# Autodesk Inventor assembly: Робот_ЕТЗ
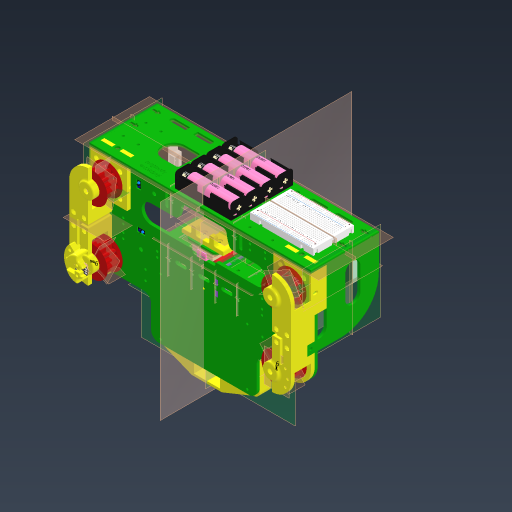
[picture p0: Inventor's stored thumbnail of the model, 512x512]
Saved by Autodesk Inventor 2023.2 (Build 272271030, 271C)
## iProperties
Created: 2025-12-08
Part Number: Робот_ЕТЗ
Document SubType Name: Assembly
Designer: Олег Коноваленко
Author: Олег Коноваленко
## Documents named in this file (25)
- D:\VSOSH_IT_Robotics_ETZ\ETZ\Сonstruction\Робот_ЕТЗ.iam
- D:\VSOSH_IT_Robotics_ETZ\ETZ\Сonstruction\Nema 17.ipt
- D:\VSOSH_IT_Robotics_ETZ\ETZ\Сonstruction\Передняя_крышка.ipt
- D:\VSOSH_IT_Robotics_ETZ\ETZ\Сonstruction\Print\Вал_ведомых_шестерн.ipt
- D:\VSOSH_IT_Robotics_ETZ\ETZ\Сonstruction\Крепление_ведомых_шестерн.ipt
- D:\VSOSH_IT_Robotics_ETZ\ETZ\Сonstruction\Фланцевая_муфта.ipt
- D:\VSOSH_IT_Robotics_ETZ\ETZ\Сonstruction\Вал_ведущих_шестерн.ipt
- D:\VSOSH_IT_Robotics_ETZ\ETZ\Сonstruction\Ведомая_шестерня.ipt
- D:\VSOSH_IT_Robotics_ETZ\ETZ\Сonstruction\Ведущая_шеестерня.ipt
- D:\VSOSH_IT_Robotics_ETZ\ETZ\Сonstruction\Крепление_ведомых_шестерн_MIR1.ipt
- D:\VSOSH_IT_Robotics_ETZ\ETZ\Сonstruction\TCRT5000.ipt
- D:\VSOSH_IT_Robotics_ETZ\ETZ\Сonstruction\Крепление_TCRT.ipt
- D:\VSOSH_IT_Robotics_ETZ\ETZ\Сonstruction\AS5048A Magnetic Encoder - B.ipt
- D:\VSOSH_IT_Robotics_ETZ\ETZ\Сonstruction\Выступ_под_крепление_маркера.ipt
- D:\VSOSH_IT_Robotics_ETZ\ETZ\Сonstruction\Рёбра_жёсткости.ipt
- D:\VSOSH_IT_Robotics_ETZ\ETZ\Сonstruction\Плата.ipt
- D:\VSOSH_IT_Robotics_ETZ\ETZ\Сonstruction\Стойка.ipt
- D:\VSOSH_IT_Robotics_ETZ\ETZ\Сonstruction\Фанерка_аккумуляторов.ipt
- D:\VSOSH_IT_Robotics_ETZ\ETZ\Сonstruction\Holder 18650 (4 cell)_series_pink.ipt
- D:\VSOSH_IT_Robotics_ETZ\ETZ\Сonstruction\Крышка_электроники.ipt
- D:\VSOSH_IT_Robotics_ETZ\ETZ\Сonstruction\Breadboard 400.ipt
- D:\VSOSH_IT_Robotics_ETZ\ETZ\Сonstruction\Крепление_энкодера.ipt
- D:\VSOSH_IT_Robotics_ETZ\ETZ\Сonstruction\Модуль_маркера.iam
- D:\VSOSH_IT_Robotics_ETZ\ETZ\Сonstruction\Рёбра_жёсткости_индивиды.ipt
- D:\VSOSH_IT_Robotics_ETZ\ETZ\Сonstruction\дополнительное_ребро_жёсткости.ipt
## Components (41 placed, 24 different names)
1. Nema 17:1 — Совмещение:78, Заподлицо:26, Угол:1
2. Передняя_крышка:1 — Совмещение:79, Совмещение:80, Совмещение:81, Заподлицо:28, Совмещение:82, Совмещение:95, Совмещение:96, Совмещение:98, Совмещение:99, Заподлицо:38, Совмещение:104, Совмещение:105, Заподлицо:42, Совмещение:109, Заподлицо:44, Заподлицо:45, Совмещение:110, Совмещение:111, Совмещение:112, Совмещение:113, Совмещение:120, Заподлицо:49, Совмещение:123, Совмещение:124, Совмещение:130, Заподлицо:57, Совмещение:143, Совмещение:144, Совмещение:145, Совмещение:146, Совмещение:147, Совмещение:148
3. Вал_ведомых_шестерн:1 — Совмещение:85
4. Крепление_ведомых_шестерн:1 — Совмещение:64, Совмещение:68, Совмещение:70, Заподлицо:23, Совмещение:73, Совмещение:79, Совмещение:80, Угол:1, Совмещение:139, Заподлицо:65, Совмещение:140, Совмещение:157, Совмещение:158
5. Фланцевая_муфта:1 — Совмещение:64, Совмещение:65, Совмещение:68, Совмещение:74, Совмещение:78, Заподлицо:26
6. Вал_ведущих_шестерн:1 — Совмещение:70, Заподлицо:23
7. Ведомая_шестерня:1 — Совмещение:85, Совмещение:157, Совмещение:158
8. Ведущая_шестерня:2 — Совмещение:65, Совмещение:73, Совмещение:74
9. Крепление_ведомых_шестерн_MIR1:1 — Совмещение:81, Заподлицо:28, Совмещение:82, Совмещение:84, Совмещение:86, Совмещение:87, Угол:2, Совмещение:119, Заподлицо:47, Заподлицо:48, Совмещение:155, Совмещение:156
10. Ведущая_шестерня:3 — Совмещение:86, Совмещение:87, Совмещение:88, Совмещение:91
11. Ведомая_шестерня:2 — Совмещение:84, Совмещение:156
12. Nema 17:2 — Совмещение:90, Заподлицо:29, Угол:2
13. Фланцевая_муфта:2 — Совмещение:88, Совмещение:90, Заподлицо:29, Совмещение:91
14. TCRT5000:1 — Совмещение:92, Заподлицо:30, Заподлицо:31
15. Крепление_TCRT:1 — Совмещение:92, Заподлицо:30, Заподлицо:31, Совмещение:95, Заподлицо:43, Заподлицо:46
16. TCRT5000:2
17. Крепление_TCRT:2 — Совмещение:96, Заподлицо:42, Заподлицо:43
18. AS5048A Magnetic Encoder - B:1 — Совмещение:136, Совмещение:137, Совмещение:138
19. Выступ_под_крепление_маркера:1 — Совмещение:98, Совмещение:99, Заподлицо:38, Совмещение:106, Совмещение:107, Совмещение:108, Заподлицо:41, Заподлицо:46, Совмещение:141, Заподлицо:66, Совмещение:142
20. Рёбра_жёсткости:3 — Совмещение:104, Совмещение:107, Совмещение:108
21. Рёбра_жёсткости:4 — Совмещение:105, Совмещение:106, Заподлицо:41
22. Плата:1 — Совмещение:109, Заподлицо:44, Заподлицо:45, Совмещение:114, Совмещение:115, Совмещение:116, Совмещение:117, Заподлицо:59, Заподлицо:60, Заподлицо:61, Заподлицо:62
23. Стойка:1 — Совмещение:110, Совмещение:115, Заподлицо:61
24. Стойка:2 — Совмещение:111, Совмещение:116, Заподлицо:62
25. Стойка:3 — Совмещение:112, Совмещение:117, Заподлицо:59
26. Стойка:4 — Совмещение:113, Совмещение:114, Заподлицо:60
27. Фанерка_аккумуляторов:1 — Совмещение:119, Заподлицо:47, Заподлицо:48, Совмещение:121, Совмещение:122, Совмещение:131, Заподлицо:63, Заподлицо:64, Совмещение:152, Заподлицо:73, Заподлицо:74, Заподлицо:75, Совмещение:154, Заподлицо:76, Заподлицо:77
28. Рёбра_жёсткости:5 — Совмещение:120, Совмещение:121, Заподлицо:49
29. Рёбра_жёсткости:6 — Совмещение:122, Совмещение:123, Совмещение:124
30. Holder 18650 (4 cell)_series_pink:1 — Заподлицо:69, Совмещение:149, Заподлицо:72
31. Holder 18650 (4 cell)_series_pink:3 — Заподлицо:68, Заподлицо:69, Совмещение:150, Совмещение:151, Заподлицо:70, Заподлицо:71, Совмещение:153
32. Holder 18650 (4 cell)_series_pink:4 — Заподлицо:67, Заподлицо:68, Совмещение:149, Совмещение:150, Заподлицо:71, Заподлицо:72
33. Крышка_электроники:1 — Совмещение:130, Заподлицо:57
34. Breadboard 400:1 — Совмещение:131, Заподлицо:63, Заподлицо:64
35. Крепление_энкодера:1 — Совмещение:136, Совмещение:137, Совмещение:138, Совмещение:139, Заподлицо:65, Совмещение:140
36. Модуль_маркера:1 [sub-assembly] — Совмещение:141, Заподлицо:66, Совмещение:142
37. Рёбра_жёсткости_индивиды:1 — Совмещение:143, Совмещение:147, Совмещение:148
38. Рёбра_жёсткости_индивиды:2 — Совмещение:144, Совмещение:145, Совмещение:146
39. Holder 18650 (4 cell)_series_pink:5 — Заподлицо:67, Совмещение:151, Заподлицо:70, Совмещение:152, Заподлицо:73
40. дополнительное_ребро_жёсткости:1 — Заподлицо:74, Заподлицо:75, Совмещение:154
41. дополнительное_ребро_жёсткости:2 — Совмещение:155, Заподлицо:76, Заподлицо:77
## Relationships (109: Mate 69, Flush 38, Angle 2)
- Совмещение:64 [Mate]: Крепление_ведомых_шестерн:1 ↔ Фланцевая_муфта:1
- Совмещение:65 [Mate]: Фланцевая_муфта:1 ↔ Ведущая_шестерня:2
- Совмещение:68 [Mate]: Крепление_ведомых_шестерн:1 ↔ Фланцевая_муфта:1
- Совмещение:70 [Mate]: Крепление_ведомых_шестерн:1 ↔ Вал_ведущих_шестерн:1
- Заподлицо:23 [Flush]: Крепление_ведомых_шестерн:1 ↔ Вал_ведущих_шестерн:1
- Совмещение:73 [Mate] (0.5 mm): Крепление_ведомых_шестерн:1 ↔ Ведущая_шестерня:2
- Совмещение:74 [Mate]: Фланцевая_муфта:1 ↔ Ведущая_шестерня:2
- Совмещение:78 [Mate]: Nema 17:1 ↔ Фланцевая_муфта:1
- Заподлицо:26 [Flush]: Nema 17:1 ↔ Фланцевая_муфта:1
- Совмещение:79 [Mate]: Передняя_крышка:1 ↔ Крепление_ведомых_шестерн:1
- Совмещение:80 [Mate]: Передняя_крышка:1 ↔ Крепление_ведомых_шестерн:1
- Совмещение:81 [Mate]: Передняя_крышка:1 ↔ Крепление_ведомых_шестерн_MIR1:1
- Заподлицо:28 [Flush]: Передняя_крышка:1 ↔ Крепление_ведомых_шестерн_MIR1:1
- Совмещение:82 [Mate]: Передняя_крышка:1 ↔ Крепление_ведомых_шестерн_MIR1:1
- Совмещение:84 [Mate]: Крепление_ведомых_шестерн_MIR1:1 ↔ Ведомая_шестерня:2
- Совмещение:85 [Mate]: Вал_ведомых_шестерн:1 ↔ Ведомая_шестерня:1
- Совмещение:86 [Mate] (0.5 mm): Крепление_ведомых_шестерн_MIR1:1 ↔ Ведущая_шестерня:3
- Совмещение:87 [Mate]: Крепление_ведомых_шестерн_MIR1:1 ↔ Ведущая_шестерня:3
- Угол:1 [Angle] (0 deg): Nema 17:1 ↔ Крепление_ведомых_шестерн:1
- Совмещение:88 [Mate]: Ведущая_шестерня:3 ↔ Фланцевая_муфта:2
- Совмещение:90 [Mate]: Nema 17:2 ↔ Фланцевая_муфта:2
- Заподлицо:29 [Flush]: Nema 17:2 ↔ Фланцевая_муфта:2
- Совмещение:91 [Mate]: Ведущая_шестерня:3 ↔ Фланцевая_муфта:2
- Угол:2 [Angle] (0 deg): Крепление_ведомых_шестерн_MIR1:1 ↔ Nema 17:2
- Совмещение:92 [Mate]: TCRT5000:1 ↔ Крепление_TCRT:1
- Заподлицо:30 [Flush]: TCRT5000:1 ↔ Крепление_TCRT:1
- Заподлицо:31 [Flush]: TCRT5000:1 ↔ Крепление_TCRT:1
- [Mate]: TCRT5000:2 ↔ Крепление_TCRT:2
- [Flush]: TCRT5000:2 ↔ Крепление_TCRT:2
- [Flush]: TCRT5000:2 ↔ Крепление_TCRT:2
- Совмещение:95 [Mate]: Передняя_крышка:1 ↔ Крепление_TCRT:1
- Совмещение:96 [Mate]: Передняя_крышка:1 ↔ Крепление_TCRT:2
- Совмещение:98 [Mate]: Передняя_крышка:1 ↔ Выступ_под_крепление_маркера:1
- Совмещение:99 [Mate]: Передняя_крышка:1 ↔ Выступ_под_крепление_маркера:1
- Заподлицо:38 [Flush] (10 mm): Передняя_крышка:1 ↔ Выступ_под_крепление_маркера:1
- Совмещение:104 [Mate]: Передняя_крышка:1 ↔ Рёбра_жёсткости:3
- Совмещение:105 [Mate]: Передняя_крышка:1 ↔ Рёбра_жёсткости:4
- Совмещение:106 [Mate]: Выступ_под_крепление_маркера:1 ↔ Рёбра_жёсткости:4
- Совмещение:107 [Mate]: Выступ_под_крепление_маркера:1 ↔ Рёбра_жёсткости:3
- Совмещение:108 [Mate] (-14.25 mm): Выступ_под_крепление_маркера:1 ↔ Рёбра_жёсткости:3
- Заподлицо:41 [Flush] (14.25 mm): Выступ_под_крепление_маркера:1 ↔ Рёбра_жёсткости:4
- Заподлицо:42 [Flush] (10 mm): Передняя_крышка:1 ↔ Крепление_TCRT:2
- Заподлицо:43 [Flush]: Крепление_TCRT:1 ↔ Крепление_TCRT:2
- Совмещение:109 [Mate] (8 mm): Передняя_крышка:1 ↔ Плата:1
- Заподлицо:44 [Flush] (10 mm): Передняя_крышка:1 ↔ Плата:1
- Заподлицо:45 [Flush] (2.75 mm): Передняя_крышка:1 ↔ Плата:1
- Совмещение:110 [Mate]: Передняя_крышка:1 ↔ Стойка:1
- Совмещение:111 [Mate]: Передняя_крышка:1 ↔ Стойка:2
- Совмещение:112 [Mate]: Передняя_крышка:1 ↔ Стойка:3
- Совмещение:113 [Mate]: Передняя_крышка:1 ↔ Стойка:4
- Совмещение:114 [Mate]: Плата:1 ↔ Стойка:4
- Совмещение:115 [Mate]: Плата:1 ↔ Стойка:1
- Совмещение:116 [Mate]: Плата:1 ↔ Стойка:2
- Совмещение:117 [Mate]: Плата:1 ↔ Стойка:3
- Заподлицо:46 [Flush]: Крепление_TCRT:1 ↔ Выступ_под_крепление_маркера:1
- Совмещение:119 [Mate]: Крепление_ведомых_шестерн_MIR1:1 ↔ Фанерка_аккумуляторов:1
- Заподлицо:47 [Flush]: Крепление_ведомых_шестерн_MIR1:1 ↔ Фанерка_аккумуляторов:1
- Заподлицо:48 [Flush]: Крепление_ведомых_шестерн_MIR1:1 ↔ Фанерка_аккумуляторов:1
- Совмещение:120 [Mate]: Передняя_крышка:1 ↔ Рёбра_жёсткости:5
- Совмещение:121 [Mate]: Фанерка_аккумуляторов:1 ↔ Рёбра_жёсткости:5
- Заподлицо:49 [Flush] (40 mm): Передняя_крышка:1 ↔ Рёбра_жёсткости:5
- Совмещение:122 [Mate]: Фанерка_аккумуляторов:1 ↔ Рёбра_жёсткости:6
- Совмещение:123 [Mate]: Передняя_крышка:1 ↔ Рёбра_жёсткости:6
- Совмещение:124 [Mate] (40 mm): Передняя_крышка:1 ↔ Рёбра_жёсткости:6
- Совмещение:130 [Mate]: Передняя_крышка:1 ↔ Крышка_электроники:1
- Заподлицо:57 [Flush]: Передняя_крышка:1 ↔ Крышка_электроники:1
- Заподлицо:59 [Flush]: Плата:1 ↔ Стойка:3
- Заподлицо:60 [Flush]: Плата:1 ↔ Стойка:4
- Заподлицо:61 [Flush]: Плата:1 ↔ Стойка:1
- Заподлицо:62 [Flush]: Плата:1 ↔ Стойка:2
- Совмещение:131 [Mate]: Фанерка_аккумуляторов:1 ↔ Breadboard 400:1
- Заподлицо:63 [Flush]: Фанерка_аккумуляторов:1 ↔ Breadboard 400:1
- Заподлицо:64 [Flush] (15 mm): Фанерка_аккумуляторов:1 ↔ Breadboard 400:1
- Совмещение:136 [Mate]: AS5048A Magnetic Encoder - B:1 ↔ Крепление_энкодера:1
- Совмещение:137 [Mate]: AS5048A Magnetic Encoder - B:1 ↔ Крепление_энкодера:1
- Совмещение:138 [Mate]: AS5048A Magnetic Encoder - B:1 ↔ Крепление_энкодера:1
- Совмещение:139 [Mate]: Крепление_ведомых_шестерн:1 ↔ Крепление_энкодера:1
- Заподлицо:65 [Flush]: Крепление_ведомых_шестерн:1 ↔ Крепление_энкодера:1
- Совмещение:140 [Mate]: Крепление_ведомых_шестерн:1 ↔ Крепление_энкодера:1
- Совмещение:141 [Mate]: Выступ_под_крепление_маркера:1 ↔ Модуль_маркера:1
- Заподлицо:66 [Flush]: Выступ_под_крепление_маркера:1 ↔ Модуль_маркера:1
- Совмещение:142 [Mate]: Выступ_под_крепление_маркера:1 ↔ Модуль_маркера:1
- Совмещение:143 [Mate]: Передняя_крышка:1 ↔ Рёбра_жёсткости_индивиды:1
- Совмещение:144 [Mate]: Передняя_крышка:1 ↔ Рёбра_жёсткости_индивиды:2
- Совмещение:145 [Mate]: Передняя_крышка:1 ↔ Рёбра_жёсткости_индивиды:2
- Совмещение:146 [Mate]: Передняя_крышка:1 ↔ Рёбра_жёсткости_индивиды:2
- Совмещение:147 [Mate]: Передняя_крышка:1 ↔ Рёбра_жёсткости_индивиды:1
- Совмещение:148 [Mate]: Передняя_крышка:1 ↔ Рёбра_жёсткости_индивиды:1
- Заподлицо:67 [Flush]: Holder 18650 (4 cell)_series_pink:4 ↔ Holder 18650 (4 cell)_series_pink:5
- Заподлицо:68 [Flush]: Holder 18650 (4 cell)_series_pink:3 ↔ Holder 18650 (4 cell)_series_pink:4
- Заподлицо:69 [Flush]: Holder 18650 (4 cell)_series_pink:1 ↔ Holder 18650 (4 cell)_series_pink:3
- Совмещение:149 [Mate]: Holder 18650 (4 cell)_series_pink:1 ↔ Holder 18650 (4 cell)_series_pink:4
- Совмещение:150 [Mate]: Holder 18650 (4 cell)_series_pink:3 ↔ Holder 18650 (4 cell)_series_pink:4
- Совмещение:151 [Mate]: Holder 18650 (4 cell)_series_pink:3 ↔ Holder 18650 (4 cell)_series_pink:5
- Заподлицо:70 [Flush]: Holder 18650 (4 cell)_series_pink:3 ↔ Holder 18650 (4 cell)_series_pink:5
- Заподлицо:71 [Flush]: Holder 18650 (4 cell)_series_pink:3 ↔ Holder 18650 (4 cell)_series_pink:4
- Заподлицо:72 [Flush]: Holder 18650 (4 cell)_series_pink:1 ↔ Holder 18650 (4 cell)_series_pink:4
- Совмещение:152 [Mate]: Фанерка_аккумуляторов:1 ↔ Holder 18650 (4 cell)_series_pink:5
- Заподлицо:73 [Flush] (4 mm): Фанерка_аккумуляторов:1 ↔ Holder 18650 (4 cell)_series_pink:5
- Совмещение:153 [Mate]: Holder 18650 (4 cell)_series_pink:3
- Заподлицо:74 [Flush]: Фанерка_аккумуляторов:1 ↔ дополнительное_ребро_жёсткости:1
- Заподлицо:75 [Flush]: Фанерка_аккумуляторов:1 ↔ дополнительное_ребро_жёсткости:1
- Совмещение:154 [Mate]: Фанерка_аккумуляторов:1 ↔ дополнительное_ребро_жёсткости:1
- Совмещение:155 [Mate]: Крепление_ведомых_шестерн_MIR1:1 ↔ дополнительное_ребро_жёсткости:2
- Заподлицо:76 [Flush]: Фанерка_аккумуляторов:1 ↔ дополнительное_ребро_жёсткости:2
- Заподлицо:77 [Flush]: Фанерка_аккумуляторов:1 ↔ дополнительное_ребро_жёсткости:2
- Совмещение:156 [Mate] (0.75 mm): Крепление_ведомых_шестерн_MIR1:1 ↔ Ведомая_шестерня:2
- Совмещение:157 [Mate] (0.75 mm): Крепление_ведомых_шестерн:1 ↔ Ведомая_шестерня:1
- Совмещение:158 [Mate]: Крепление_ведомых_шестерн:1 ↔ Ведомая_шестерня:1
## Named parameters: d165_d160 = 0 mm, d166_d161 = 0 mm, d167_d162 = 0 mm
